# Autodesk Inventor assembly: lane_floor
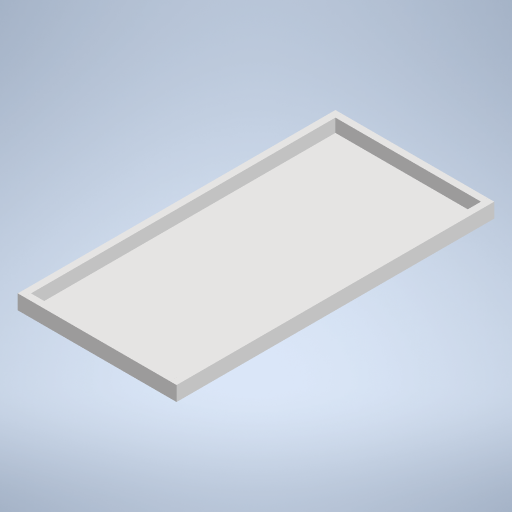
[picture p0: Inventor's stored thumbnail of the model, 512x512]
Saved by Autodesk Inventor 2024.2 (Build 282272000, 272)
## iProperties
Created: 2024-01-12
Part Number: lane_floor
Document SubType Name: Assembly
Designer: nicky
Author: nicky
## Documents named in this file (4)
- E:\OneDrive - 성균관대학교\Projects\2024 ICRA QRC 대회\모델\lane_floor.iam
- E:\OneDrive - 성균관대학교\Projects\2024 ICRA QRC 대회\모델\board_2400x1200x11.ipt
- E:\OneDrive - 성균관대학교\Projects\2024 ICRA QRC 대회\모델\board_50x100x2400.ipt
- E:\OneDrive - 성균관대학교\Projects\2024 ICRA QRC 대회\모델\board_50x100x1100.ipt
## Components (5 placed, 3 different names)
1. board_2400x1200x11:1 — 플러쉬:1, 플러쉬:2, 강체:1, 플러쉬:3, 플러쉬:4, 메이트:1
2. board_50x100x2400:1 — 플러쉬:1, 플러쉬:2
3. board_50x100x2400:2 — 강체:1, 메이트:2, 플러쉬:5
4. board_50x100x1100:1 — 플러쉬:3, 플러쉬:4
5. board_50x100x1100:2 — 메이트:1, 메이트:2, 플러쉬:5
## Relationships (8: Flush 5, Mate 2, WeldJoint 1)
- 플러쉬:1 [Flush]: board_2400x1200x11:1 ↔ board_50x100x2400:1
- 플러쉬:2 [Flush]: board_2400x1200x11:1 ↔ board_50x100x2400:1
- 강체:1 [WeldJoint]: board_2400x1200x11:1 ↔ board_50x100x2400:2
- 플러쉬:3 [Flush]: board_2400x1200x11:1 ↔ board_50x100x1100:1
- 플러쉬:4 [Flush]: board_2400x1200x11:1 ↔ board_50x100x1100:1
- 메이트:1 [Mate]: board_2400x1200x11:1 ↔ board_50x100x1100:2
- 메이트:2 [Mate]: board_50x100x2400:2 ↔ board_50x100x1100:2
- 플러쉬:5 [Flush]: board_50x100x2400:2 ↔ board_50x100x1100:2
